# Autodesk Inventor assembly: FarmBot
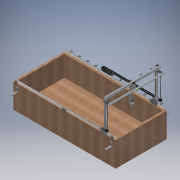
[picture p0: Inventor's stored thumbnail of the model, 180x180]
Saved by Autodesk Inventor 2017 (Build 210142000, 142)
## iProperties
Created: 2016-12-12
Part Number: FarmBot
Document SubType Name: Assembly
Designer: umr
Author: umr
## Documents named in this file (19)
- C:\Users\Ali\Desktop\roboticFarm-master\Models2\FarmBot.iam
- C:\Users\Ali\Desktop\roboticFarm-master\Models2\BedAssembly\BedAseembly.iam
- C:\Users\Ali\Desktop\roboticFarm-master\Models2\Head\HeadSlider.iam
- C:\Users\Ali\Desktop\roboticFarm-master\Models2\Gantry\GantryDown.iam
- C:\Users\Ali\Desktop\roboticFarm-master\Models2\Gantry\GantryUp.iam
- C:\Users\Ali\Desktop\roboticFarm-master\Models2\Case\Case.iam
- C:\Users\Ali\Desktop\roboticFarm-master\Models2\CableCarier\Tracks Drag Chain Assembly.iam
- C:\Users\Ali\Desktop\roboticFarm-master\Models2\CableCarier\Tee Nut.ipt
- C:\Users\Ali\Desktop\roboticFarm-master\Models2\CableCarier\Track Joining Plate_MIR.ipt
- C:\Users\Ali\Desktop\roboticFarm-master\Models2\CableCarier\M5 Screw_MIR.ipt
- C:\Users\Ali\Desktop\roboticFarm-master\Models2\CableCarier\Wood Screw 99136A600_MIR.ipt
- C:\Users\Ali\Desktop\roboticFarm-master\Models2\CableCarier\Track Joining Plate_MIR_MIR.ipt
- C:\Users\Ali\Desktop\roboticFarm-master\Models2\CableCarier\M5 Screw_MIR_MIR.ipt
- C:\Users\Ali\Desktop\roboticFarm-master\Models2\CableCarier\Wood Screw 99136A600_MIR_MIR.ipt
- C:\Users\Ali\Desktop\roboticFarm-master\Models2\CableCarier\Tee Nut_MIR.ipt
- C:\Users\Ali\Desktop\roboticFarm-master\Models2\CableCarier\Drag Chain Support Bracket with Tee Nut.iam
- C:\Users\Ali\Desktop\roboticFarm-master\Models2\CableCarier\Drag Chain Support Bracket with Tee Nut_MIR.iam
- C:\Users\Ali\Desktop\roboticFarm-master\Models2\CableCarier\Tracks Drag Chain Assembly_MIR.iam
- C:\Users\Ali\Desktop\roboticFarm-master\Models2\Gantry\GantryDown_MIR.iam
## Components (58 placed, 18 different names)
1. BedAseembly:2 [sub-assembly] — Mate:9, Tangent:1, Tangent:2, Mate:10, Mate:11, Mate:12, Mate:13, Flush:1, Mate:17, Mate:18
2. HeadSlider:1 [sub-assembly] — Mate:6, Mate:7
3. GantryDown:1 [sub-assembly] — Mate:3, Mate:5, Mate:9, Tangent:1, Tangent:2
4. GantryUp:1 [sub-assembly] — Mate:3, Mate:5, Mate:6, Mate:7
5. Case:1 [sub-assembly] — Mate:10, Mate:11, Mate:12, Mate:13
6. Tracks Drag Chain Assembly:1 [sub-assembly] — Mate:19
7. Drag Chain Support Bracket with Tee Nut_MIR:1 [sub-assembly]
8. Drag Chain Support Bracket with Tee Nut_MIR:2 [sub-assembly]
9. Drag Chain Support Bracket with Tee Nut_MIR:3 [sub-assembly]
10. Drag Chain Support Bracket with Tee Nut_MIR:4 [sub-assembly]
11. Drag Chain Support Bracket with Tee Nut_MIR:5 [sub-assembly]
12. Drag Chain Support Bracket with Tee Nut_MIR:6 [sub-assembly]
13. Drag Chain Support Bracket with Tee Nut_MIR:7 [sub-assembly]
14. Drag Chain Support Bracket with Tee Nut_MIR:8 [sub-assembly]
15. Drag Chain Support Bracket with Tee Nut_MIR:9 [sub-assembly]
16. Drag Chain Support Bracket with Tee Nut_MIR:10 [sub-assembly]
17. Drag Chain Support Bracket with Tee Nut_MIR:11 [sub-assembly]
18. Drag Chain Support Bracket with Tee Nut_MIR:12 [sub-assembly]
19. Tracks Drag Chain Assembly_MIR:1 [sub-assembly]
20. GantryDown_MIR:1 [sub-assembly]
21. Track Joining Plate_MIR:1 — Rigid:19, Rigid:20, Rigid:21, Rigid:22, Rigid:23, Rigid:24, Rigid:25, Rigid:26, Insert:4, Insert:6, Insert:7, Insert:8, Mate:17
22. M5 Screw_MIR:1 — Rigid:25
23. M5 Screw_MIR:2 — Rigid:24
24. M5 Screw_MIR:3 — Rigid:23
25. Wood Screw 99136A600_MIR:1 — Rigid:20
26. Wood Screw 99136A600_MIR:2 — Rigid:19
27. Wood Screw 99136A600_MIR:3 — Rigid:21
28. Wood Screw 99136A600_MIR:4 — Rigid:22
29. M5 Screw_MIR:4 — Rigid:26
30. Tee Nut:12 — Insert:4
31. Tee Nut:13 — Insert:6
32. Tee Nut:14 — Insert:8
33. Tee Nut:15 — Insert:7
34. Track Joining Plate_MIR_MIR:1 — Insert:9, Insert:10, Insert:11, Insert:12, Rigid:27, Rigid:28, Rigid:29, Rigid:30, Rigid:31, Rigid:32, Rigid:33, Rigid:34
35. M5 Screw_MIR_MIR:1 — Rigid:27
36. M5 Screw_MIR_MIR:2 — Rigid:28
37. M5 Screw_MIR_MIR:3 — Rigid:29
38. Wood Screw 99136A600_MIR_MIR:1 — Rigid:30
39. Wood Screw 99136A600_MIR_MIR:2 — Rigid:31
40. Wood Screw 99136A600_MIR_MIR:3 — Rigid:32
41. Wood Screw 99136A600_MIR_MIR:4 — Rigid:33
42. M5 Screw_MIR_MIR:4 — Rigid:34
43. Tee Nut_MIR:1 — Insert:9
44. Tee Nut_MIR:2 — Insert:10
45. Tee Nut_MIR:3 — Insert:11
46. Tee Nut_MIR:4 — Insert:12
47. Drag Chain Support Bracket with Tee Nut:2 [sub-assembly] — Mate:18
48. Drag Chain Support Bracket with Tee Nut:3 [sub-assembly]
49. Drag Chain Support Bracket with Tee Nut:4 [sub-assembly]
50. Drag Chain Support Bracket with Tee Nut:5 [sub-assembly]
51. Drag Chain Support Bracket with Tee Nut:6 [sub-assembly]
52. Drag Chain Support Bracket with Tee Nut:7 [sub-assembly] — Mate:19
53. Drag Chain Support Bracket with Tee Nut:8 [sub-assembly]
54. Drag Chain Support Bracket with Tee Nut:9 [sub-assembly]
55. Drag Chain Support Bracket with Tee Nut:10 [sub-assembly]
56. Drag Chain Support Bracket with Tee Nut:11 [sub-assembly]
57. Drag Chain Support Bracket with Tee Nut:12 [sub-assembly]
58. Drag Chain Support Bracket with Tee Nut:13 [sub-assembly]
## Component patterns: (12 elements, first: Drag Chain Support Bracket with Tee Nut:2)
## Relationships (39: WeldJoint 16, Mate 12, Insert 8, Tangent 2, Flush 1)
- Mate:3: GantryDown:1 ↔ GantryUp:1
- Mate:5: GantryDown:1 ↔ GantryUp:1
- Mate:6: HeadSlider:1 ↔ GantryUp:1
- Mate:7: HeadSlider:1 ↔ GantryUp:1
- Mate:9: BedAseembly:2 ↔ GantryDown:1
- Tangent:1: BedAseembly:2 ↔ GantryDown:1
- Tangent:2: BedAseembly:2 ↔ GantryDown:1
- Mate:10: BedAseembly:2 ↔ Case:1
- Mate:11: BedAseembly:2 ↔ Case:1
- Mate:12: BedAseembly:2 ↔ Case:1
- Mate:13: BedAseembly:2 ↔ Case:1
- Flush:1 (575 mm): BedAseembly:2
- Rigid:19 [WeldJoint]: Track Joining Plate_MIR:1 ↔ Wood Screw 99136A600_MIR:2
- Rigid:20 [WeldJoint]: Track Joining Plate_MIR:1 ↔ Wood Screw 99136A600_MIR:1
- Rigid:21 [WeldJoint]: Track Joining Plate_MIR:1 ↔ Wood Screw 99136A600_MIR:3
- Rigid:22 [WeldJoint]: Track Joining Plate_MIR:1 ↔ Wood Screw 99136A600_MIR:4
- Rigid:23 [WeldJoint]: Track Joining Plate_MIR:1 ↔ M5 Screw_MIR:3
- Rigid:24 [WeldJoint]: Track Joining Plate_MIR:1 ↔ M5 Screw_MIR:2
- Rigid:25 [WeldJoint]: Track Joining Plate_MIR:1 ↔ M5 Screw_MIR:1
- Rigid:26 [WeldJoint]: Track Joining Plate_MIR:1 ↔ M5 Screw_MIR:4
- Insert:4: Track Joining Plate_MIR:1 ↔ Tee Nut:12
- Insert:6: Track Joining Plate_MIR:1 ↔ Tee Nut:13
- Insert:7: Track Joining Plate_MIR:1 ↔ Tee Nut:15
- Insert:8: Track Joining Plate_MIR:1 ↔ Tee Nut:14
- Mate:17: BedAseembly:2 ↔ Track Joining Plate_MIR:1
- Insert:9: Track Joining Plate_MIR_MIR:1 ↔ Tee Nut_MIR:1
- Insert:10: Track Joining Plate_MIR_MIR:1 ↔ Tee Nut_MIR:2
- Insert:11: Track Joining Plate_MIR_MIR:1 ↔ Tee Nut_MIR:3
- Insert:12: Track Joining Plate_MIR_MIR:1 ↔ Tee Nut_MIR:4
- Rigid:27 [WeldJoint]: Track Joining Plate_MIR_MIR:1 ↔ M5 Screw_MIR_MIR:1
- Rigid:28 [WeldJoint]: Track Joining Plate_MIR_MIR:1 ↔ M5 Screw_MIR_MIR:2
- Rigid:29 [WeldJoint]: Track Joining Plate_MIR_MIR:1 ↔ M5 Screw_MIR_MIR:3
- Rigid:30 [WeldJoint]: Track Joining Plate_MIR_MIR:1 ↔ Wood Screw 99136A600_MIR_MIR:1
- Rigid:31 [WeldJoint]: Track Joining Plate_MIR_MIR:1 ↔ Wood Screw 99136A600_MIR_MIR:2
- Rigid:32 [WeldJoint]: Track Joining Plate_MIR_MIR:1 ↔ Wood Screw 99136A600_MIR_MIR:3
- Rigid:33 [WeldJoint]: Track Joining Plate_MIR_MIR:1 ↔ Wood Screw 99136A600_MIR_MIR:4
- Rigid:34 [WeldJoint]: Track Joining Plate_MIR_MIR:1 ↔ M5 Screw_MIR_MIR:4
- Mate:18: BedAseembly:2 ↔ Drag Chain Support Bracket with Tee Nut:2
- Mate:19: Tracks Drag Chain Assembly:1 ↔ Drag Chain Support Bracket with Tee Nut:7
